# Autodesk Inventor assembly: beercart assembly - mekatronik backup
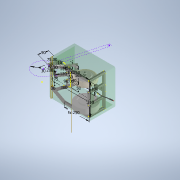
[picture p0: Inventor's stored thumbnail of the model, 180x180]
Saved by Autodesk Inventor 2022.2 (Build 262287000, 287)
## iProperties
_SolveAssemblyDoc: Frame Generator Solve Assembly
_Version: 15.0.0
Created: 2022-03-11
Part Number: beercart assembly - mekatronik backup
Document SubType Name: Assembly
Designer: foriw
Mass: 9394.64 g
Surface Area: 15952.6 cm^2
Volume: 7017.96 cm^3
Density: 1.33866 g/cm^3
Author: foriw
## Documents named in this file (9)
- C:\Users\foriw\OneDrive\Dokumenter\Inventor\Beercart - Meaktroronik - new\Mekatronik-beerCart\beercart assembly - mekatronik backup.iam
- C:\Users\foriw\OneDrive\Dokumenter\Inventor\Beercart - Meaktroronik - new\beercart- framwork - baseSketch.ipt
- C:\Users\foriw\OneDrive\Dokumenter\Inventor\Beercart - Meaktroronik - new\beercart assembly - mekatronik\Frame\Frame 1647030135921.iam
- C:\Users\foriw\OneDrive\Dokumenter\Inventor\Beercart - Meaktroronik - new\8 inch wheel assembly.ipt
- C:\Users\foriw\OneDrive\Dokumenter\Inventor\Beercart - Meaktroronik - new\motor at24v.ipt
- C:\Users\foriw\OneDrive\Dokumenter\Inventor\Beercart - Meaktroronik - new\beer crate.ipt
- C:\Users\foriw\OneDrive\Dokumenter\Inventor\Beercart - Meaktroronik - new\bearing housing front.ipt
- C:\Users\foriw\OneDrive\Dokumenter\Inventor\Beercart - Meaktroronik - new\bearing housing front_MIR.ipt
- C:\Users\foriw\OneDrive\Dokumenter\Inventor\adaptive tire project - physics exame\frontwheel frame.ipt
## Components (8 placed, 8 different names)
1. beercart- framwork - baseSketch:1
2. Frame 1647030135921:1 [sub-assembly] — Mate:1, Flush:1, Flush:3
3. 8 inch wheel assembly:1
4. motor at24v:1
5. beer crate:1 — Flush:2, Flush:3
6. bearing housing front:1 — Mate:1, Flush:1
7. bearing housing front_MIR:1
8. frontwheel frame:1
## Relationships (4: Flush 3, Mate 1)
- Mate:1: Frame 1647030135921:1 ↔ bearing housing front:1
- Flush:1 (1 mm): Frame 1647030135921:1 ↔ bearing housing front:1
- Flush:2: beer crate:1
- Flush:3: Frame 1647030135921:1 ↔ beer crate:1
